# Autodesk Inventor assembly: BC-100005
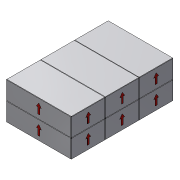
[picture p0: Inventor's stored thumbnail of the model, 180x180]
Saved by Autodesk Inventor 2016 (Build 200138000, 138)
## iProperties
Created: 2015-10-05
Part Number: BC-100005
Document SubType Name: Assembly
Designer: Insira seu nome aqui!
Author: Insira seu nome aqui!
## Documents named in this file (2)
- D:\ARQ\Basilio\LNLS-2\Anel\Dipolos\BC-3T\Dipolo 3T e 1T\Prototipo 1\Projeto Mecanico\BC-100005.iam
- D:\ARQ\Basilio\LNLS-2\Anel\Dipolos\BC-3T\Dipolo 3T e 1T\Prototipo 1\Projeto Mecanico\NdFeB.ipt
## Components (6 placed, 1 different names)
1. NdFeB:1 — Mate:2, Flush:1, Flush:2, Flush:4, Flush:6, Flush:7, Mate:4
2. NdFeB:2 — Mate:3, Flush:2, Flush:5, Flush:7, Mate:4, Flush:8
3. NdFeB:3 — Mate:1, Flush:1, Flush:3, Flush:6, Flush:9
4. NdFeB:4 — Mate:1, Flush:3, Flush:9, Mate:5
5. NdFeB:5 — Mate:2, Flush:4, Mate:5
6. NdFeB:6 — Mate:3, Flush:5, Flush:8
## Relationships (14: Flush 9, Mate 5)
- Mate:1: NdFeB:3 ↔ NdFeB:4
- Mate:2: NdFeB:1 ↔ NdFeB:5
- Mate:3: NdFeB:2 ↔ NdFeB:6
- Flush:1: NdFeB:1 ↔ NdFeB:3
- Flush:2: NdFeB:1 ↔ NdFeB:2
- Flush:3: NdFeB:3 ↔ NdFeB:4
- Flush:4: NdFeB:1 ↔ NdFeB:5
- Flush:5: NdFeB:2 ↔ NdFeB:6
- Flush:6: NdFeB:1 ↔ NdFeB:3
- Flush:7: NdFeB:1 ↔ NdFeB:2
- Mate:4: NdFeB:1 ↔ NdFeB:2
- Flush:8: NdFeB:2 ↔ NdFeB:6
- Flush:9: NdFeB:3 ↔ NdFeB:4
- Mate:5: NdFeB:4 ↔ NdFeB:5
